# Autodesk Inventor assembly: Robot
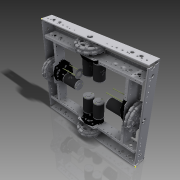
[picture p0: Inventor's stored thumbnail of the model, 180x180]
Saved by Autodesk Inventor 2015 (Build 190159000, 159)
## iProperties
Created: 2015-01-10
Part Number: Robot
Document SubType Name: Assembly
Designer: jhirshland1
Author: jhirshland1
## Documents named in this file (9)
- C:\Users\jhirshland1\Inventor\HWRobot2015\Chassis.iam
- C:\Users\jhirshland1\Inventor\HWRobot2015\FRCKOP2015\Drive Base\am-2951 AM14U2 Outside Sheet.ipt
- C:\Users\jhirshland1\Inventor\HWRobot2015\Frame\Corner of Frame.iam
- C:\Users\jhirshland1\Inventor\HWRobot2015\FRCKOP2015\Drive Base\am-2951 AM14U2 Ouside resized for 201.ipt
- C:\Users\jhirshland1\Inventor\HWRobot2015\FRCKOP2015\Drive Base\am-2951 AM14U2 Ouside 23i.ipt
- C:\Users\jhirshland1\Inventor\HWRobot2015\FRCKOP2015\Drive Base\Aluminum Mount Plate.ipt
- C:\Users\jhirshland1\Inventor\HWRobot2015\FRCKOP2015\Drive Base\am-2952 AM14U2 Inside Sheet.ipt
- C:\Users\jhirshland1\Inventor\HWRobot2015\FRCKOP2015\AndyMark\WheelAssembly.iam
- C:\Users\jhirshland1\Inventor\HWRobot2015\FRCKOP2015\AndyMark\SecondWheelAssembl.iam
## Components (13 placed, 8 different names)
1. Corner of Frame:1 [sub-assembly]
2. am-2951 AM14U2 Ouside resized for 201:1
3. am-2951 AM14U2 Outside Sheet:1 — Mate:1, Flush:1, Mate:5, Mate:8, Mate:15
4. Aluminum Mount Plate:1 — Mate:1, Flush:1, Flush:4, Mate:4, Flush:5, Flush:6, Flush:7, Mate:6, Flush:8, Flush:10, Mate:7, Mate:11, Mate:14
5. am-2951 AM14U2 Outside Sheet:2 — Flush:4, Mate:4, Flush:5, Flush:6, Mate:16
6. am-2951 AM14U2 Ouside 23i:1 — Flush:7, Mate:5, Mate:6, Mate:19
7. am-2951 AM14U2 Ouside 23i:2 — Flush:8, Flush:10, Mate:7, Mate:8, Mate:13, Mate:17, Mate:21
8. am-2952 AM14U2 Inside Sheet:1 — Mate:11, Mate:16, Mate:17, Mate:18, Mate:20, Flush:11, Flush:12
9. am-2952 AM14U2 Inside Sheet:2 — Mate:13, Mate:14, Mate:15, Insert:3, Insert:4
10. WheelAssembly:1 [sub-assembly]
11. WheelAssembly:2 [sub-assembly] — Insert:3, Insert:4
12. SecondWheelAssembl:1 [sub-assembly] — Mate:18, Mate:19, Flush:12
13. SecondWheelAssembl:2 [sub-assembly] — Mate:20, Flush:11, Mate:21
## Relationships (29: Mate 16, Flush 9, Insert 4)
- Mate:1: am-2951 AM14U2 Outside Sheet:1 ↔ Aluminum Mount Plate:1
- Flush:1: am-2951 AM14U2 Outside Sheet:1 ↔ Aluminum Mount Plate:1
- Flush:4: Aluminum Mount Plate:1 ↔ am-2951 AM14U2 Outside Sheet:2
- Mate:4: Aluminum Mount Plate:1 ↔ am-2951 AM14U2 Outside Sheet:2
- Flush:5: Aluminum Mount Plate:1 ↔ am-2951 AM14U2 Outside Sheet:2
- Flush:6: Aluminum Mount Plate:1 ↔ am-2951 AM14U2 Outside Sheet:2
- Flush:7: Aluminum Mount Plate:1 ↔ am-2951 AM14U2 Ouside 23i:1
- Mate:5: am-2951 AM14U2 Outside Sheet:1 ↔ am-2951 AM14U2 Ouside 23i:1
- Mate:6: Aluminum Mount Plate:1 ↔ am-2951 AM14U2 Ouside 23i:1
- Flush:8: Aluminum Mount Plate:1 ↔ am-2951 AM14U2 Ouside 23i:2
- Flush:10: Aluminum Mount Plate:1 ↔ am-2951 AM14U2 Ouside 23i:2
- Mate:7: Aluminum Mount Plate:1 ↔ am-2951 AM14U2 Ouside 23i:2
- Mate:8: am-2951 AM14U2 Outside Sheet:1 ↔ am-2951 AM14U2 Ouside 23i:2
- Mate:11: Aluminum Mount Plate:1 ↔ am-2952 AM14U2 Inside Sheet:1
- Mate:13: am-2951 AM14U2 Ouside 23i:2 ↔ am-2952 AM14U2 Inside Sheet:2
- Mate:14: Aluminum Mount Plate:1 ↔ am-2952 AM14U2 Inside Sheet:2
- Mate:15 (85.09 mm): am-2951 AM14U2 Outside Sheet:1 ↔ am-2952 AM14U2 Inside Sheet:2
- Mate:16 (85.09 mm): am-2951 AM14U2 Outside Sheet:2 ↔ am-2952 AM14U2 Inside Sheet:1
- Mate:17: am-2951 AM14U2 Ouside 23i:2 ↔ am-2952 AM14U2 Inside Sheet:1
- [Insert]: am-2952 AM14U2 Inside Sheet:1 ↔ WheelAssembly:1
- [Insert]: am-2952 AM14U2 Inside Sheet:1 ↔ WheelAssembly:1
- Insert:3: am-2952 AM14U2 Inside Sheet:2 ↔ WheelAssembly:2
- Insert:4: am-2952 AM14U2 Inside Sheet:2 ↔ WheelAssembly:2
- Mate:18: am-2952 AM14U2 Inside Sheet:1 ↔ SecondWheelAssembl:1
- Mate:19 (85.09 mm): am-2951 AM14U2 Ouside 23i:1 ↔ SecondWheelAssembl:1
- Mate:20: am-2952 AM14U2 Inside Sheet:1 ↔ SecondWheelAssembl:2
- Flush:11: am-2952 AM14U2 Inside Sheet:1 ↔ SecondWheelAssembl:2
- Mate:21 (85.09 mm): am-2951 AM14U2 Ouside 23i:2 ↔ SecondWheelAssembl:2
- Flush:12: am-2952 AM14U2 Inside Sheet:1 ↔ SecondWheelAssembl:1
